# Autodesk Inventor assembly: Assembly1
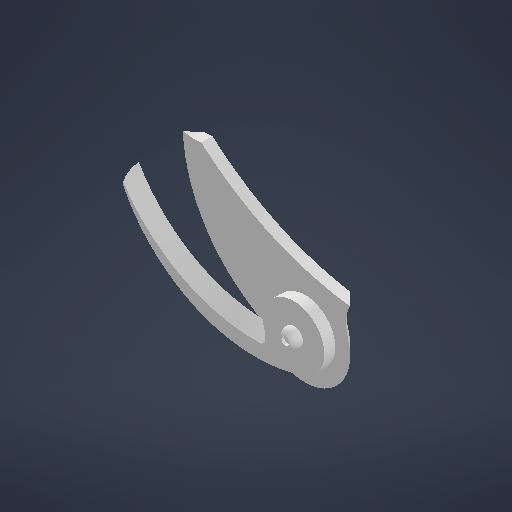
[picture p0: Inventor's stored thumbnail of the model, 512x512]
Saved by Autodesk Inventor 2026.1 (Build 301233020, 233B)
## iProperties
Created: 2025-11-05
Part Number: Assembly1
Document SubType Name: Assembly
Designer: Marcelo
Author: Marcelo
## Documents named in this file (4)
- C:\Users\Marcelo\OneDrive\Documents\GitHub\proyecto-integrador\Assembly1.iam
- C:\Users\Marcelo\OneDrive\Documents\GitHub\proyecto-integrador\Hoja de Corte.ipt
- C:\Users\Marcelo\OneDrive\Documents\GitHub\proyecto-integrador\Contrahoja.ipt
- C:\Users\Marcelo\OneDrive\Documents\GitHub\proyecto-integrador\Perno.ipt
## Components (3 placed, 3 different names)
1. Hoja de Corte:1 — Rotational:2
2. Contrahoja:1 — Rotational:1
3. Perno:1 — Rotational:1, Rotational:2
## Relationships (2: RevoluteJoint 2)
- Rotational:1 [RevoluteJoint] (-7 mm): Contrahoja:1 ↔ Perno:1
- Rotational:2 [RevoluteJoint] (-4 mm): Hoja de Corte:1 ↔ Perno:1
